# Autodesk Inventor assembly: Intake Pivot Assembly
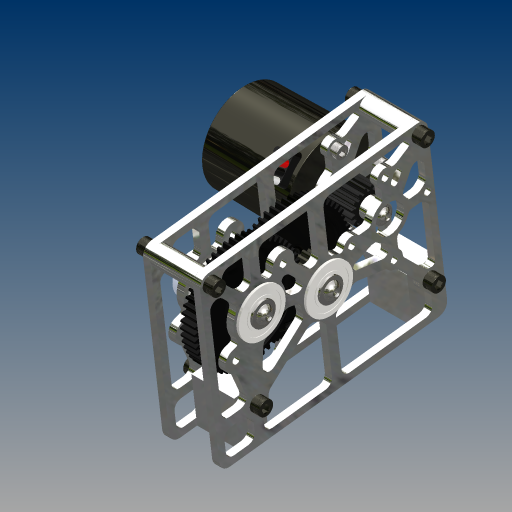
[picture p0: Inventor's stored thumbnail of the model, 512x512]
Saved by Autodesk Inventor 2024.3 (Build 283343000, 343)
## iProperties
Created: 2024-08-01
Part Number: Intake Pivot Assembly
Document SubType Name: Assembly
Designer: Kenji
Author: Kenji
## Documents named in this file (21)
- C:\Users\Kenji\Documents\GitHub\1622-2024-Summer-CAD-A-Thon\Intake\Intake Pivot Assembly.iam
- C:\Users\Kenji\Documents\GitHub\1622-2024-Summer-CAD-A-Thon\COTS Library\Motors\COTS_REV-21-1650-V1.1_Neo1.1.ipt
- C:\Users\Kenji\Documents\GitHub\1622-2024-Summer-CAD-A-Thon\Intake\WCP-1236 (1).ipt
- C:\Users\Kenji\Documents\GitHub\1622-2024-Summer-CAD-A-Thon\COTS Library\Motion\Bearings\COTS_WCP-0783_1.125ODHexBearing.ipt
- C:\Users\Kenji\Documents\GitHub\1622-2024-Summer-CAD-A-Thon\COTS Library\Fasteners\Bolts\Socket-Head\10-32\COTS_91251A340__3-18in long_Black-Oxide Alloy Steel Socket Head.ipt
- C:\Users\Kenji\Documents\GitHub\1622-2024-Summer-CAD-A-Thon\Intake\Intake Pivot Spacer 1.ipt
- C:\Users\Kenji\Documents\GitHub\1622-2024-Summer-CAD-A-Thon\Intake\Intake Pivot Spacer 2.ipt
- C:\Users\Kenji\Documents\GitHub\1622-2024-Summer-CAD-A-Thon\Intake\Intake Pivot Hex Shaft.ipt
- C:\Users\Kenji\Documents\GitHub\1622-2024-Summer-CAD-A-Thon\Intake\Intake Pivot Spacer 3.ipt
- C:\Users\Kenji\Documents\GitHub\1622-2024-Summer-CAD-A-Thon\COTS Library\Fasteners\Bolts\Socket-Head\0.25-20\COTS_91251A537_Black-Oxide Alloy Steel Socket Head Screw.ipt
- C:\Users\Kenji\Documents\GitHub\1622-2024-Summer-CAD-A-Thon\COTS Library\Fasteners\Washers\COTS_90107A029_316 Stainless Steel Washer.ipt
- C:\Users\Kenji\Documents\GitHub\1622-2024-Summer-CAD-A-Thon\COTS Library\Fasteners\Washers\COTS_91860A047_Size10Washer.ipt
- C:\Users\Kenji\Documents\GitHub\1622-2024-Summer-CAD-A-Thon\COTS Library\Fasteners\Bolts\Button-Head\10-32\COTS_92949A265_1-2in long Stainless Steel Button Head Screw.ipt
- C:\Users\Kenji\Documents\GitHub\1622-2024-Summer-CAD-A-Thon\Intake\Intake Pivot Gearbox Plate.ipt
- C:\Users\Kenji\Documents\GitHub\1622-2024-Summer-CAD-A-Thon\COTS Library\Motion\Gears\20DP gears\Steel\0.5in hex\COTS_WCP-0733_Steel_18T20DPGear.ipt
- C:\Users\Kenji\Documents\GitHub\1622-2024-Summer-CAD-A-Thon\Intake\WCP-0185.ipt
- C:\Users\Kenji\Documents\GitHub\1622-2024-Summer-CAD-A-Thon\Intake\WCP-0184.ipt
- C:\Users\Kenji\Documents\GitHub\1622-2024-Summer-CAD-A-Thon\COTS Library\Fasteners\Bolts\Button-Head\0.25-20\COTS_0.25-20_ButtonHead_0.5inlong_StainlessSteel_92949A537.ipt
- C:\Users\Kenji\Documents\GitHub\1622-2024-Summer-CAD-A-Thon\Intake\Intake Pivot Billet.ipt
- C:\Users\Kenji\Documents\GitHub\1622-2024-Summer-CAD-A-Thon\COTS Library\Fasteners\Bolts\Socket-Head\0.25-20\COTS_91251A539_Black-Oxide Alloy Steel Socket Head Screw (1).ipt
- C:\Users\Kenji\Documents\GitHub\1622-2024-Summer-CAD-A-Thon\COTS Library\Fasteners\Shaft Collars\COTS_WCP-0799_0.5inchHexShaftCollar.ipt
## Components (39 placed, 20 different names)
1. COTS_REV-21-1650-V1.1_Neo1.1:1 — Mate:6, Mate:33, Mate:63, Mate:75, Mate:96, Mate:97
2. WCP-1236 (1):1 — Mate:6, Mate:34, Mate:80
3. COTS_WCP-0783_1.125ODHexBearing:1 — Flush:3, Mate:56, Mate:85, Mate:86, Flush:4, Mate:111, Mate:112, Mate:113, Mate:127, Mate:128
4. COTS_WCP-0783_1.125ODHexBearing:2 — Mate:81, Mate:82, Mate:98, Mate:108, Mate:109, Mate:133
5. COTS_WCP-0783_1.125ODHexBearing:3 — Mate:60, Mate:87, Mate:88, Flush:4, Mate:114, Mate:115, Mate:142, Mate:143
6. COTS_WCP-0783_1.125ODHexBearing:4 — Mate:83, Mate:84, Mate:110
7. COTS_91251A340__3-18in long_Black-Oxide Alloy Steel Socket Head:2 — Mate:100, Mate:104
8. COTS_91251A340__3-18in long_Black-Oxide Alloy Steel Socket Head:4 — Mate:99, Mate:103
9. COTS_91251A340__3-18in long_Black-Oxide Alloy Steel Socket Head:6 — Mate:101, Mate:102
10. Intake Pivot Spacer 1:1 — Mate:33, Mate:34, Mate:76
11. Intake Pivot Spacer 2:1 — Mate:113, Mate:114, Mate:115
12. Intake Pivot Hex Shaft:2 — Flush:3, Mate:59, Mate:117
13. Intake Pivot Spacer 3:2 — Mate:89, Mate:90, Mate:91, Mate:92, Mate:93
14. COTS_91251A537_Black-Oxide Alloy Steel Socket Head Screw:1 — Mate:90, Mate:94
15. COTS_91251A537_Black-Oxide Alloy Steel Socket Head Screw:2 — Mate:89, Mate:95
16. COTS_91251A537_Black-Oxide Alloy Steel Socket Head Screw:7 — Mate:57, Mate:58, Mate:59, Mate:98
17. COTS_90107A029_316 Stainless Steel Washer:1 — Mate:56, Mate:116, Mate:117, Mate:118
18. COTS_90107A029_316 Stainless Steel Washer:2 — Mate:57, Mate:58, Mate:60
19. COTS_91860A047_Size10Washer:1 — Mate:61, Mate:62, Mate:63, Mate:76
20. COTS_92949A265_1-2in long Stainless Steel Button Head Screw:1 — Mate:61, Mate:62
21. Intake Pivot Gearbox Plate:1 — Mate:73, Mate:74, Mate:81, Mate:82, Mate:85, Mate:86, Mate:91, Mate:92, Mate:94, Mate:120, Mate:121, Mate:124, Mate:129, Mate:130, Mate:135, Mate:137, Mate:138, Mate:141
22. Intake Pivot Gearbox Plate:2 — Mate:73, Mate:74, Mate:75, Mate:80, Mate:83, Mate:84, Mate:87, Mate:88, Mate:93, Mate:95, Mate:96, Mate:97, Mate:99, Mate:100, Mate:101, Mate:102, Mate:103, Mate:104, Mate:105, Mate:106, Mate:119, Mate:122, Mate:123, Mate:131, Mate:132, Flush:5, Flush:6, Mate:134, Mate:136, Mate:139, Mate:140
23. COTS_91251A340__3-18in long_Black-Oxide Alloy Steel Socket Head:7 — Mate:105, Mate:106
24. COTS_WCP-0733_Steel_18T20DPGear:1 — Mate:108, Mate:133
25. WCP-0185:1 — Mate:109, Mate:110
26. WCP-0184:1 — Mate:111, Mate:112
27. COTS_0.25-20_ButtonHead_0.5inlong_StainlessSteel_92949A537:1 — Mate:116, Mate:118
28. Intake Pivot Spacer 3:3 — Mate:119, Mate:120
29. COTS_91251A537_Black-Oxide Alloy Steel Socket Head Screw:8 — Mate:121, Mate:124
30. COTS_91251A537_Black-Oxide Alloy Steel Socket Head Screw:9 — Mate:122, Mate:123
31. COTS_0.25-20_ButtonHead_0.5inlong_StainlessSteel_92949A537:2 — Mate:125, Mate:126
32. COTS_90107A029_316 Stainless Steel Washer:4 — Mate:125, Mate:126, Mate:127, Mate:128
33. Intake Pivot Billet:1 — Mate:129, Mate:132, Flush:5
34. Intake Pivot Billet:2 — Mate:130, Mate:131, Flush:6
35. COTS_91251A539_Black-Oxide Alloy Steel Socket Head Screw (1):1 — Mate:134, Mate:136
36. COTS_91251A539_Black-Oxide Alloy Steel Socket Head Screw (1):2 — Mate:135, Mate:137
37. COTS_91251A539_Black-Oxide Alloy Steel Socket Head Screw (1):3 — Mate:138, Mate:141
38. COTS_91251A539_Black-Oxide Alloy Steel Socket Head Screw (1):4 — Mate:139, Mate:140
39. COTS_WCP-0799_0.5inchHexShaftCollar:1 — Mate:142, Mate:143
## Relationships (82: Mate 78, Flush 4)
- Mate:6: COTS_REV-21-1650-V1.1_Neo1.1:1 ↔ WCP-1236 (1):1
- Mate:33: COTS_REV-21-1650-V1.1_Neo1.1:1 ↔ Intake Pivot Spacer 1:1
- Mate:34: WCP-1236 (1):1 ↔ Intake Pivot Spacer 1:1
- Flush:3: COTS_WCP-0783_1.125ODHexBearing:1 ↔ Intake Pivot Hex Shaft:2
- Mate:56: COTS_WCP-0783_1.125ODHexBearing:1 ↔ COTS_90107A029_316 Stainless Steel Washer:1
- Mate:57: COTS_91251A537_Black-Oxide Alloy Steel Socket Head Screw:7 ↔ COTS_90107A029_316 Stainless Steel Washer:2
- Mate:58: COTS_91251A537_Black-Oxide Alloy Steel Socket Head Screw:7 ↔ COTS_90107A029_316 Stainless Steel Washer:2
- Mate:59: Intake Pivot Hex Shaft:2 ↔ COTS_91251A537_Black-Oxide Alloy Steel Socket Head Screw:7
- Mate:60: COTS_WCP-0783_1.125ODHexBearing:3 ↔ COTS_90107A029_316 Stainless Steel Washer:2
- Mate:61: COTS_91860A047_Size10Washer:1 ↔ COTS_92949A265_1-2in long Stainless Steel Button Head Screw:1
- Mate:62: COTS_91860A047_Size10Washer:1 ↔ COTS_92949A265_1-2in long Stainless Steel Button Head Screw:1
- Mate:63: COTS_REV-21-1650-V1.1_Neo1.1:1 ↔ COTS_91860A047_Size10Washer:1
- Mate:73: Intake Pivot Gearbox Plate:1 ↔ Intake Pivot Gearbox Plate:2
- Mate:74: Intake Pivot Gearbox Plate:1 ↔ Intake Pivot Gearbox Plate:2
- Mate:75: COTS_REV-21-1650-V1.1_Neo1.1:1 ↔ Intake Pivot Gearbox Plate:2
- Mate:76: Intake Pivot Spacer 1:1 ↔ COTS_91860A047_Size10Washer:1
- Mate:80: WCP-1236 (1):1 ↔ Intake Pivot Gearbox Plate:2
- Mate:81: COTS_WCP-0783_1.125ODHexBearing:2 ↔ Intake Pivot Gearbox Plate:1
- Mate:82: COTS_WCP-0783_1.125ODHexBearing:2 ↔ Intake Pivot Gearbox Plate:1
- Mate:83: COTS_WCP-0783_1.125ODHexBearing:4 ↔ Intake Pivot Gearbox Plate:2
- Mate:84: COTS_WCP-0783_1.125ODHexBearing:4 ↔ Intake Pivot Gearbox Plate:2
- Mate:85: COTS_WCP-0783_1.125ODHexBearing:1 ↔ Intake Pivot Gearbox Plate:1
- Mate:86: COTS_WCP-0783_1.125ODHexBearing:1 ↔ Intake Pivot Gearbox Plate:1
- Mate:87: COTS_WCP-0783_1.125ODHexBearing:3 ↔ Intake Pivot Gearbox Plate:2
- Mate:88: COTS_WCP-0783_1.125ODHexBearing:3 ↔ Intake Pivot Gearbox Plate:2
- Mate:89: Intake Pivot Spacer 3:2 ↔ COTS_91251A537_Black-Oxide Alloy Steel Socket Head Screw:2
- Mate:90: Intake Pivot Spacer 3:2 ↔ COTS_91251A537_Black-Oxide Alloy Steel Socket Head Screw:1
- Mate:91: Intake Pivot Spacer 3:2 ↔ Intake Pivot Gearbox Plate:1
- Mate:92: Intake Pivot Spacer 3:2 ↔ Intake Pivot Gearbox Plate:1
- Mate:93: Intake Pivot Spacer 3:2 ↔ Intake Pivot Gearbox Plate:2
- Mate:94: COTS_91251A537_Black-Oxide Alloy Steel Socket Head Screw:1 ↔ Intake Pivot Gearbox Plate:1
- Mate:95: COTS_91251A537_Black-Oxide Alloy Steel Socket Head Screw:2 ↔ Intake Pivot Gearbox Plate:2
- Mate:96: COTS_REV-21-1650-V1.1_Neo1.1:1 ↔ Intake Pivot Gearbox Plate:2
- Mate:97: COTS_REV-21-1650-V1.1_Neo1.1:1 ↔ Intake Pivot Gearbox Plate:2
- Mate:98: COTS_WCP-0783_1.125ODHexBearing:2 ↔ COTS_91251A537_Black-Oxide Alloy Steel Socket Head Screw:7
- Mate:99: COTS_91251A340__3-18in long_Black-Oxide Alloy Steel Socket Head:4 ↔ Intake Pivot Gearbox Plate:2
- Mate:100: COTS_91251A340__3-18in long_Black-Oxide Alloy Steel Socket Head:2 ↔ Intake Pivot Gearbox Plate:2
- Mate:101: COTS_91251A340__3-18in long_Black-Oxide Alloy Steel Socket Head:6 ↔ Intake Pivot Gearbox Plate:2
- Mate:102: COTS_91251A340__3-18in long_Black-Oxide Alloy Steel Socket Head:6 ↔ Intake Pivot Gearbox Plate:2
- Mate:103: COTS_91251A340__3-18in long_Black-Oxide Alloy Steel Socket Head:4 ↔ Intake Pivot Gearbox Plate:2
- Mate:104: COTS_91251A340__3-18in long_Black-Oxide Alloy Steel Socket Head:2 ↔ Intake Pivot Gearbox Plate:2
- Mate:105: Intake Pivot Gearbox Plate:2 ↔ COTS_91251A340__3-18in long_Black-Oxide Alloy Steel Socket Head:7
- Mate:106: Intake Pivot Gearbox Plate:2 ↔ COTS_91251A340__3-18in long_Black-Oxide Alloy Steel Socket Head:7
- Mate:108: COTS_WCP-0783_1.125ODHexBearing:2 ↔ COTS_WCP-0733_Steel_18T20DPGear:1
- Mate:109: COTS_WCP-0783_1.125ODHexBearing:2 ↔ WCP-0185:1
- Mate:110: COTS_WCP-0783_1.125ODHexBearing:4 ↔ WCP-0185:1
- Flush:4: COTS_WCP-0783_1.125ODHexBearing:1 ↔ COTS_WCP-0783_1.125ODHexBearing:3
- Mate:111: COTS_WCP-0783_1.125ODHexBearing:1 ↔ WCP-0184:1
- Mate:112: COTS_WCP-0783_1.125ODHexBearing:1 ↔ WCP-0184:1
- Mate:113: COTS_WCP-0783_1.125ODHexBearing:1 ↔ Intake Pivot Spacer 2:1
- Mate:114: COTS_WCP-0783_1.125ODHexBearing:3 ↔ Intake Pivot Spacer 2:1
- Mate:115: COTS_WCP-0783_1.125ODHexBearing:3 ↔ Intake Pivot Spacer 2:1
- Mate:116: COTS_90107A029_316 Stainless Steel Washer:1 ↔ COTS_0.25-20_ButtonHead_0.5inlong_StainlessSteel_92949A537:1
- Mate:117: Intake Pivot Hex Shaft:2 ↔ COTS_90107A029_316 Stainless Steel Washer:1
- Mate:118: COTS_90107A029_316 Stainless Steel Washer:1 ↔ COTS_0.25-20_ButtonHead_0.5inlong_StainlessSteel_92949A537:1
- Mate:119: Intake Pivot Gearbox Plate:2 ↔ Intake Pivot Spacer 3:3
- Mate:120: Intake Pivot Gearbox Plate:1 ↔ Intake Pivot Spacer 3:3
- Mate:121: Intake Pivot Gearbox Plate:1 ↔ COTS_91251A537_Black-Oxide Alloy Steel Socket Head Screw:8
- Mate:122: Intake Pivot Gearbox Plate:2 ↔ COTS_91251A537_Black-Oxide Alloy Steel Socket Head Screw:9
- Mate:123: Intake Pivot Gearbox Plate:2 ↔ COTS_91251A537_Black-Oxide Alloy Steel Socket Head Screw:9
- Mate:124: Intake Pivot Gearbox Plate:1 ↔ COTS_91251A537_Black-Oxide Alloy Steel Socket Head Screw:8
- Mate:125: COTS_0.25-20_ButtonHead_0.5inlong_StainlessSteel_92949A537:2 ↔ COTS_90107A029_316 Stainless Steel Washer:4
- Mate:126: COTS_0.25-20_ButtonHead_0.5inlong_StainlessSteel_92949A537:2 ↔ COTS_90107A029_316 Stainless Steel Washer:4
- Mate:127: COTS_WCP-0783_1.125ODHexBearing:1 ↔ COTS_90107A029_316 Stainless Steel Washer:4
- Mate:128: COTS_WCP-0783_1.125ODHexBearing:1 ↔ COTS_90107A029_316 Stainless Steel Washer:4
- Mate:129: Intake Pivot Gearbox Plate:1 ↔ Intake Pivot Billet:1
- Mate:130: Intake Pivot Gearbox Plate:1 ↔ Intake Pivot Billet:2
- Mate:131: Intake Pivot Gearbox Plate:2 ↔ Intake Pivot Billet:2
- Mate:132: Intake Pivot Gearbox Plate:2 ↔ Intake Pivot Billet:1
- Flush:5: Intake Pivot Gearbox Plate:2 ↔ Intake Pivot Billet:1
- Flush:6: Intake Pivot Gearbox Plate:2 ↔ Intake Pivot Billet:2
- Mate:133: COTS_WCP-0783_1.125ODHexBearing:2 ↔ COTS_WCP-0733_Steel_18T20DPGear:1
- Mate:134: Intake Pivot Gearbox Plate:2 ↔ COTS_91251A539_Black-Oxide Alloy Steel Socket Head Screw (1):1
- Mate:135: Intake Pivot Gearbox Plate:1 ↔ COTS_91251A539_Black-Oxide Alloy Steel Socket Head Screw (1):2
- Mate:136: Intake Pivot Gearbox Plate:2 ↔ COTS_91251A539_Black-Oxide Alloy Steel Socket Head Screw (1):1
- Mate:137: Intake Pivot Gearbox Plate:1 ↔ COTS_91251A539_Black-Oxide Alloy Steel Socket Head Screw (1):2
- Mate:138: Intake Pivot Gearbox Plate:1 ↔ COTS_91251A539_Black-Oxide Alloy Steel Socket Head Screw (1):3
- Mate:139: Intake Pivot Gearbox Plate:2 ↔ COTS_91251A539_Black-Oxide Alloy Steel Socket Head Screw (1):4
- Mate:140: Intake Pivot Gearbox Plate:2 ↔ COTS_91251A539_Black-Oxide Alloy Steel Socket Head Screw (1):4
- Mate:141: Intake Pivot Gearbox Plate:1 ↔ COTS_91251A539_Black-Oxide Alloy Steel Socket Head Screw (1):3
- Mate:142: COTS_WCP-0783_1.125ODHexBearing:3 ↔ COTS_WCP-0799_0.5inchHexShaftCollar:1
- Mate:143: COTS_WCP-0783_1.125ODHexBearing:3 ↔ COTS_WCP-0799_0.5inchHexShaftCollar:1
